# Autodesk Inventor assembly: Sun_TrainOnStraightTrack
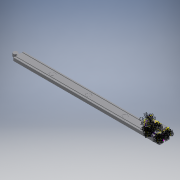
[picture p0: Inventor's stored thumbnail of the model, 180x180]
Saved by Autodesk Inventor 2016 (Build 200138000, 138)
## iProperties
Created: 2018-01-31
Part Number: Sun_TrainOnStraightTrack
Document SubType Name: Assembly
Designer: sun01147
Author: sun01147
## Documents named in this file (11)
- E:\IED7_SunT\IED7_ToyTrain\Sun_TrainOnStraightTrack.iam
- E:\IED7_SunT\IED7_ToyTrain\Sun_EngineBody.ipt
- E:\IED7_SunT\IED7_ToyTrain\HitchMagnet.ipt
- E:\IED7_SunT\IED7_ToyTrain\Linkage Peg.ipt
- E:\IED7_SunT\IED7_ToyTrain\Sun_CowCatcher.ipt
- E:\IED7_SunT\IED7_ToyTrain\Sun_wheel.ipt
- E:\IED7_SunT\IED7_ToyTrain\Sun_AxlePeg.ipt
- E:\IED7_SunT\IED7_ToyTrain\Sun_Stack.ipt
- E:\IED7_SunT\IED7_ToyTrain\HitchPeg.ipt
- E:\IED7_SunT\IED7_ToyTrain\Sun_LinkageArm.ipt
- E:\IED7_SunT\IED7_ToyTrain\Sun_StraightTrack.ipt
## Components (23 placed, 11 different names)
1. Sun_EngineBody:1 — Mate:1, Mate:2, Mate:4, Angle:1, Mate:22, Insert:2, Insert:3, Insert:4, Insert:5, Insert:16, Insert:17, Insert:18, Angle:2, Angle:3, Drive Angle, Mate:29, Flush:4, DriveForwardFlush
2. HitchMagnet:1 — Mate:22, Insert:18, Insert:19
3. Sun_Stack:1 — Mate:1, Mate:2, Mate:4, Angle:1
4. HitchPeg:1 — Insert:19
5. Linkage Peg:2 — Insert:12
6. Sun_wheel:3 — Insert:2, Insert:8, Mate:24, Angle:4
7. Sun_wheel:4 — Insert:3, Insert:9, Insert:11
8. Sun_AxlePeg:5 — Insert:8
9. Sun_AxlePeg:6 — Insert:6
10. Sun_AxlePeg:7 — Insert:7
11. Sun_wheel Drive — Insert:5, Insert:7, Mate:25, Insert:12, Drive Angle
12. Sun_wheel:7 — Insert:4, Insert:6, Insert:10, Angle:4
13. Sun_AxlePeg:8 — Insert:9
14. Sun_LinkageArm:1 — Insert:10, Mate:25, Insert:13, Angle:2
15. Sun_LinkageArm:2 — Insert:11, Mate:24, Insert:14, Insert:15, Angle:3
16. Linkage Peg:3 — Insert:13
17. Linkage Peg:4 — Insert:14
18. Linkage Peg:5 — Insert:15
19. Sun_CowCatcher:1 — Insert:16, Insert:17
20. Sun_StraightTrack:1 — Mate:27, Mate:28
21. Sun_StraightTrack:2 — Flush:1, Flush:3, Mate:26, Mate:27, Mate:29, Flush:4
22. Sun_StraightTrack:3 — Flush:1, Flush:2, Flush:3, Mate:26
23. Sun_StraightTrack:4 — Flush:2, Mate:28, DriveForwardFlush
## Relationships (38: Insert 18, Mate 10, Angle 5, Flush 5)
- Mate:1: Sun_EngineBody:1 ↔ Sun_Stack:1
- Mate:2: Sun_EngineBody:1 ↔ Sun_Stack:1
- Mate:4: Sun_EngineBody:1 ↔ Sun_Stack:1
- Angle:1 (0 deg): Sun_EngineBody:1 ↔ Sun_Stack:1
- Mate:22: Sun_EngineBody:1 ↔ HitchMagnet:1
- Insert:2 (0.254 mm): Sun_EngineBody:1 ↔ Sun_wheel:3
- Insert:3 (0.254 mm): Sun_EngineBody:1 ↔ Sun_wheel:4
- Insert:4 (0.254 mm): Sun_EngineBody:1 ↔ Sun_wheel:7
- Insert:5: Sun_EngineBody:1 ↔ Sun_wheel Drive
- Insert:6 (0.254 mm): Sun_AxlePeg:6 ↔ Sun_wheel:7
- Insert:7 (0.254 mm): Sun_AxlePeg:7 ↔ Sun_wheel Drive
- Insert:8 (0.254 mm): Sun_wheel:3 ↔ Sun_AxlePeg:5
- Insert:9 (0.254 mm): Sun_wheel:4 ↔ Sun_AxlePeg:8
- Insert:10 (0.254 mm): Sun_wheel:7 ↔ Sun_LinkageArm:1
- Insert:11 (0.254 mm): Sun_wheel:4 ↔ Sun_LinkageArm:2
- Mate:24: Sun_wheel:3 ↔ Sun_LinkageArm:2
- Mate:25: Sun_wheel Drive ↔ Sun_LinkageArm:1
- Insert:12 (0.254 mm): Linkage Peg:2 ↔ Sun_wheel Drive
- Insert:13 (0.254 mm): Sun_LinkageArm:1 ↔ Linkage Peg:3
- Insert:14 (0.254 mm): Sun_LinkageArm:2 ↔ Linkage Peg:4
- Insert:15 (0.254 mm): Sun_LinkageArm:2 ↔ Linkage Peg:5
- Insert:16: Sun_EngineBody:1 ↔ Sun_CowCatcher:1
- Insert:17: Sun_EngineBody:1 ↔ Sun_CowCatcher:1
- Insert:18: Sun_EngineBody:1 ↔ HitchMagnet:1
- Insert:19: HitchMagnet:1 ↔ HitchPeg:1
- Angle:2 (0 deg): Sun_EngineBody:1 ↔ Sun_LinkageArm:1
- Angle:3 (0 deg): Sun_EngineBody:1 ↔ Sun_LinkageArm:2
- Angle:4 (180 deg): Sun_wheel:3 ↔ Sun_wheel:7
- Drive Angle [Angle] (0 deg): Sun_EngineBody:1 ↔ Sun_wheel Drive
- Flush:1: Sun_StraightTrack:2 ↔ Sun_StraightTrack:3
- Flush:2: Sun_StraightTrack:3 ↔ Sun_StraightTrack:4
- Flush:3: Sun_StraightTrack:2 ↔ Sun_StraightTrack:3
- Mate:26: Sun_StraightTrack:2 ↔ Sun_StraightTrack:3
- Mate:27: Sun_StraightTrack:1 ↔ Sun_StraightTrack:2
- Mate:28: Sun_StraightTrack:1 ↔ Sun_StraightTrack:4
- Mate:29 (10.16 mm): Sun_EngineBody:1 ↔ Sun_StraightTrack:2
- Flush:4 (17.78 mm): Sun_EngineBody:1 ↔ Sun_StraightTrack:2
- DriveForwardFlush [Flush]: Sun_EngineBody:1 ↔ Sun_StraightTrack:4
## Named parameters: Angle = 0 deg
